# Autodesk Inventor assembly: Assembly3
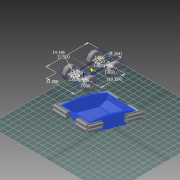
[picture p0: Inventor's stored thumbnail of the model, 180x180]
Saved by Autodesk Inventor 2015 (Build 190159000, 159)
## iProperties
Created: 2016-01-18
Part Number: Assembly3
Document SubType Name: Assembly
Designer: sethbattis
Author: sethbattis
## Documents named in this file (4)
- \\area51\team3566\cad\FRC 2016\Space Claims.iam
- \\area51\team3566\cad\FRC 2016\Basic Frame.ipt
- \\area51\team3566\cad\FRC 2016\Corner Bumper.ipt
- \\area51\team3566\cad\FRC 2016\Wheel Orientation.iam
## Components (6 placed, 3 different names)
1. Basic Frame:1 — Mate:7, Mate:8, Flush:4, Mate:9, Flush:5, Mate:10, Mate:11, Flush:6, Mate:12, Mate:13, Flush:7, Mate:14
2. Wheel Orientation:1 [sub-assembly]
3. Corner Bumper:1 — Mate:9, Flush:5, Mate:10
4. Corner Bumper:2 — Mate:11, Flush:6, Mate:12
5. Corner Bumper:3 — Mate:13, Flush:7, Mate:14
6. Corner Bumper:4 — Mate:7, Mate:8, Flush:4
## Relationships (12: Mate 8, Flush 4)
- Mate:7: Basic Frame:1 ↔ Corner Bumper:4
- Mate:8: Basic Frame:1 ↔ Corner Bumper:4
- Flush:4: Basic Frame:1 ↔ Corner Bumper:4
- Mate:9: Basic Frame:1 ↔ Corner Bumper:1
- Flush:5: Basic Frame:1 ↔ Corner Bumper:1
- Mate:10: Basic Frame:1 ↔ Corner Bumper:1
- Mate:11: Basic Frame:1 ↔ Corner Bumper:2
- Flush:6: Basic Frame:1 ↔ Corner Bumper:2
- Mate:12: Basic Frame:1 ↔ Corner Bumper:2
- Mate:13: Basic Frame:1 ↔ Corner Bumper:3
- Flush:7: Basic Frame:1 ↔ Corner Bumper:3
- Mate:14: Basic Frame:1 ↔ Corner Bumper:3
